# Autodesk Inventor assembly: PowerUnit_MTM_Tool_Assembly
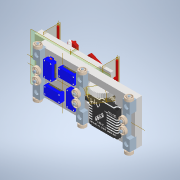
[picture p0: Inventor's stored thumbnail of the model, 180x180]
Saved by Autodesk Inventor 2022 (Build 260153000, 153)
## iProperties
Created: 2022-08-02
Part Number: PowerUnit_MTM_Tool_Assembly
Document SubType Name: Assembly
Designer: alexw
Author: alexw
## Documents named in this file (11)
- C:\Users\alexw\Documents\Inventor\Projects\03_CurrentProjects\MasterThesis\PSM_V1_Rillenkugellager\Ueberarbeiteter DaVincikopf\PowerUnit_MTM_Tool_Assembly.iam
- C:\Users\alexw\Documents\Inventor\Projects\03_CurrentProjects\MasterThesis\PSM_V1_Rillenkugellager\Ueberarbeiteter DaVincikopf\Fuehrungsgrundplatte_V3.ipt
- C:\Users\alexw\Documents\Inventor\Projects\03_CurrentProjects\MasterThesis\PSM_V1_Rillenkugellager\Ueberarbeiteter DaVincikopf\JX BLS-HV7146MG.iam
- C:\Users\alexw\Documents\Inventor\Projects\03_CurrentProjects\MasterThesis\PSM_V1_Rillenkugellager\Ueberarbeiteter DaVincikopf\SG90 - Micro Servo 9g - Tower Pro.iam
- C:\Users\alexw\Documents\Inventor\Projects\03_CurrentProjects\MasterThesis\PSM_V1_Rillenkugellager\Ueberarbeiteter DaVincikopf\Fuehrungslagerhalter_v2.ipt
- C:\Users\alexw\Documents\Inventor\Projects\03_CurrentProjects\MasterThesis\PSM_V1_Rillenkugellager\Ueberarbeiteter DaVincikopf\Adaptation_on_OPdevside_4_2.ipt
- C:\Users\alexw\Documents\Inventor\Projects\03_CurrentProjects\MasterThesis\PSM_V1_Rillenkugellager\Ueberarbeiteter DaVincikopf\Lager.iam
- C:\Users\alexw\Documents\Inventor\Projects\03_CurrentProjects\MasterThesis\PSM_V1_Rillenkugellager\Ueberarbeiteter DaVincikopf\Zahnrad.ipt
- C:\Users\alexw\Documents\Inventor\Projects\03_CurrentProjects\MasterThesis\PSM_V1_Rillenkugellager\Ueberarbeiteter DaVincikopf\Oberteil_servoplatte.ipt
- C:\Users\alexw\Documents\Inventor\Projects\03_CurrentProjects\MasterThesis\PSM_V1_Rillenkugellager\Ueberarbeiteter DaVincikopf\Adaptation_2.ipt
- C:\Users\alexw\Documents\Inventor\Projects\03_CurrentProjects\MasterThesis\PSM_V1_Rillenkugellager\Ueberarbeiteter DaVincikopf\Adaptation_2_1.ipt
## Components (29 placed, 10 different names)
1. Fuehrungsgrundplatte_V3:1 — Passend:24, Fluchtend:6, Fluchtend:7
2. JX BLS-HV7146MG:1 [sub-assembly]
3. SG90 - Micro Servo 9g - Tower Pro:1 [sub-assembly]
4. SG90 - Micro Servo 9g - Tower Pro:2 [sub-assembly]
5. SG90 - Micro Servo 9g - Tower Pro:3 [sub-assembly]
6. SG90 - Micro Servo 9g - Tower Pro:4 [sub-assembly]
7. Fuehrungslagerhalter_v2:1
8. Fuehrungslagerhalter_v2:2
9. Fuehrungslagerhalter_v2:3
10. Adaptation_on_OPdevside_4_2:1
11. Adaptation_on_OPdevside_4_2:2
12. Adaptation_on_OPdevside_4_2:3
13. Adaptation_on_OPdevside_4_2:4
14. Lager:1 [sub-assembly]
15. Lager:2 [sub-assembly]
16. Lager:3 [sub-assembly]
17. Lager:4 [sub-assembly]
18. Lager:5 [sub-assembly]
19. Lager:6 [sub-assembly]
20. Lager:7 [sub-assembly]
21. Lager:8 [sub-assembly]
22. Lager:9 [sub-assembly]
23. Lager:10 [sub-assembly]
24. Lager:11 [sub-assembly]
25. Lager:12 [sub-assembly]
26. Zahnrad:1
27. Oberteil_servoplatte:1
28. Adaptation_2:1
29. Adaptation_2_1:1
## Relationships (51: Mate 24, RevoluteJoint 17, Flush 7, Insert 3)
- [Flush] (-5 mm): Fuehrungsgrundplatte_V3:1 ↔ JX BLS-HV7146MG:1
- [Mate]: Fuehrungsgrundplatte_V3:1 ↔ JX BLS-HV7146MG:1
- [Mate]: Fuehrungsgrundplatte_V3:1 ↔ JX BLS-HV7146MG:1
- [Mate]: Fuehrungsgrundplatte_V3:1 ↔ SG90 - Micro Servo 9g - Tower Pro:4
- [Mate]: Fuehrungsgrundplatte_V3:1 ↔ SG90 - Micro Servo 9g - Tower Pro:2
- [Mate]: Fuehrungsgrundplatte_V3:1 ↔ SG90 - Micro Servo 9g - Tower Pro:3
- [Mate]: Fuehrungsgrundplatte_V3:1 ↔ SG90 - Micro Servo 9g - Tower Pro:1
- [Mate] (0.5 mm): Fuehrungsgrundplatte_V3:1 ↔ SG90 - Micro Servo 9g - Tower Pro:3
- [Mate] (0.5 mm): Fuehrungsgrundplatte_V3:1 ↔ SG90 - Micro Servo 9g - Tower Pro:3
- [Mate] (0.5 mm): Fuehrungsgrundplatte_V3:1 ↔ SG90 - Micro Servo 9g - Tower Pro:2
- [Mate] (0.5 mm): Fuehrungsgrundplatte_V3:1 ↔ SG90 - Micro Servo 9g - Tower Pro:2
- [Mate] (0.5 mm): Fuehrungsgrundplatte_V3:1 ↔ SG90 - Micro Servo 9g - Tower Pro:1
- [Mate] (0.5 mm): Fuehrungsgrundplatte_V3:1 ↔ SG90 - Micro Servo 9g - Tower Pro:1
- [Mate] (0.5 mm): Fuehrungsgrundplatte_V3:1 ↔ SG90 - Micro Servo 9g - Tower Pro:4
- [Mate] (0.5 mm): Fuehrungsgrundplatte_V3:1 ↔ SG90 - Micro Servo 9g - Tower Pro:4
- [Mate]: Fuehrungsgrundplatte_V3:1 ↔ Fuehrungslagerhalter_v2:1
- [Mate]: Fuehrungsgrundplatte_V3:1 ↔ Fuehrungslagerhalter_v2:1
- [Flush]: Fuehrungsgrundplatte_V3:1 ↔ Fuehrungslagerhalter_v2:1
- [Mate]: Fuehrungsgrundplatte_V3:1 ↔ Fuehrungslagerhalter_v2:2
- [Flush]: Fuehrungsgrundplatte_V3:1 ↔ Fuehrungslagerhalter_v2:2
- [Mate]: Fuehrungsgrundplatte_V3:1 ↔ Fuehrungslagerhalter_v2:2
- [Mate]: Fuehrungsgrundplatte_V3:1 ↔ Fuehrungslagerhalter_v2:3
- [Flush]: Fuehrungsgrundplatte_V3:1 ↔ Fuehrungslagerhalter_v2:3
- [Mate]: Fuehrungsgrundplatte_V3:1 ↔ Fuehrungslagerhalter_v2:3
- [RevoluteJoint]: Fuehrungslagerhalter_v2:1 ↔ Lager:10
- [RevoluteJoint]: Fuehrungslagerhalter_v2:2 ↔ Lager:11
- [RevoluteJoint]: Fuehrungslagerhalter_v2:3 ↔ Lager:12
- [RevoluteJoint]: Fuehrungslagerhalter_v2:3 ↔ Lager:9
- [RevoluteJoint]: Fuehrungslagerhalter_v2:2 ↔ Lager:8
- [RevoluteJoint]: Fuehrungslagerhalter_v2:1 ↔ Lager:7
- [RevoluteJoint]: Fuehrungslagerhalter_v2:3 ↔ Lager:5
- [RevoluteJoint]: Fuehrungslagerhalter_v2:3 ↔ Lager:6
- [RevoluteJoint]: Fuehrungslagerhalter_v2:2 ↔ Lager:3
- [RevoluteJoint]: Fuehrungslagerhalter_v2:2 ↔ Lager:4
- [RevoluteJoint]: Fuehrungslagerhalter_v2:1 ↔ Lager:1
- [RevoluteJoint]: Fuehrungslagerhalter_v2:1 ↔ Lager:2
- [RevoluteJoint]: JX BLS-HV7146MG:1 ↔ Zahnrad:1
- [RevoluteJoint]: SG90 - Micro Servo 9g - Tower Pro:3 ↔ Adaptation_on_OPdevside_4_2:4
- [RevoluteJoint]: SG90 - Micro Servo 9g - Tower Pro:4 ↔ Adaptation_on_OPdevside_4_2:3
- [RevoluteJoint]: SG90 - Micro Servo 9g - Tower Pro:1 ↔ Adaptation_on_OPdevside_4_2:1
- [RevoluteJoint]: SG90 - Micro Servo 9g - Tower Pro:2 ↔ Adaptation_on_OPdevside_4_2:2
- [Mate]: Fuehrungsgrundplatte_V3:1 ↔ Oberteil_servoplatte:1
- [Flush]: Fuehrungsgrundplatte_V3:1 ↔ Oberteil_servoplatte:1
- [Insert]: Fuehrungsgrundplatte_V3:1 ↔ Oberteil_servoplatte:1
- [Insert] (-5 mm): Oberteil_servoplatte:1 ↔ Adaptation_2:1
- [Mate]: Oberteil_servoplatte:1 ↔ Adaptation_2:1
- [Insert] (-5 mm): Oberteil_servoplatte:1 ↔ Adaptation_2_1:1
- [Mate]: Oberteil_servoplatte:1 ↔ Adaptation_2_1:1
- Passend:24 [Mate]: Fuehrungsgrundplatte_V3:1
- Fluchtend:6 [Flush]: Fuehrungsgrundplatte_V3:1
- Fluchtend:7 [Flush]: Fuehrungsgrundplatte_V3:1
## Named parameters: d15_d52 = 0 mm, d16_d53 = 2.715479 deg, d17_d54 = 0 mm, d18_d55 = 2.715479 deg, d19_d60 = 0 mm, d20_d61 = 101.787871 deg, d21_d32 = 0 mm, d22_d33 = 4.121163 deg, d23_d34 = 0 mm, d24_d35 = 4.121163 deg, d25_d36 = 0 mm, d26_d37 = 4.121163 deg, d27_d38 = 0 mm, d28_d39 = -4.121163 deg, d29_d40 = 0 mm, d30_d41 = -4.121163 deg, d31_d42 = 0 mm, d32_d43 = -4.121163 deg, d33_d44 = 0 mm, d34_d45 = 2.715479 deg, d35_d46 = 0 mm, d36_d47 = 2.715479 deg, d37_d48 = 0 mm, d38_d49 = 2.715479 deg, d39_d50 = 0 mm, d40_d51 = 2.715479 deg
